# Autodesk Inventor assembly: enc-BackPanel Top - Assembly
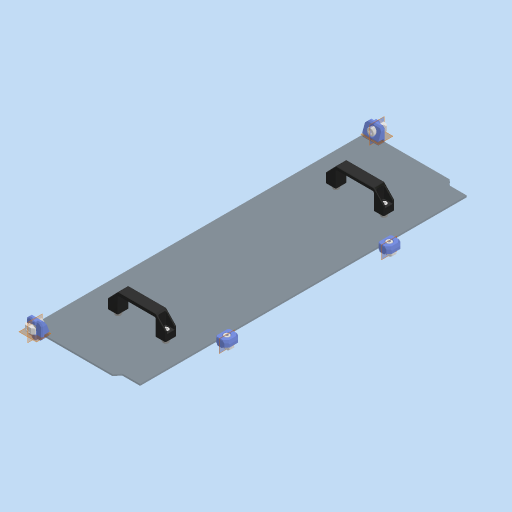
[picture p0: Inventor's stored thumbnail of the model, 512x512]
Saved by Autodesk Inventor 2023.2 (Build 272271000, 271)
## iProperties
Created: 2023-12-04
Part Number: enc-BackPanel Top - Assembly
Document SubType Name: Assembly
Designer: Nils Bade
Author: Nils Bade
## Documents named in this file (7)
- C:\Users\nilsb\Documents\Inventor\Projektarbeit-Bade\Enclosure\enc-BackPanel Top - Assembly.iam
- C:\Users\nilsb\Documents\Inventor\Projektarbeit-Bade\Enclosure\enc-BackPanel Top.ipt
- C:\Users\nilsb\Documents\Inventor\Projektarbeit-Bade\Enclosure\V-Slot Door Handle v1.ipt
- C:\Users\nilsb\Documents\Inventor\Projektarbeit-Bade\Schrauben\Cap Head Screw M6x16 - DIN912.ipt
- C:\Users\nilsb\Documents\Inventor\Projektarbeit-Bade\RatRig_Standards\Hex Locking Nut - M6 v2.ipt
- C:\Users\nilsb\Documents\Inventor\Projektarbeit-Bade\Enclosure\Panel Mount Vertical Support for 4040 - Assembly.iam
- C:\Users\nilsb\Documents\Inventor\Projektarbeit-Bade\Enclosure\Panel Mount Vertical Guide for 4040 - Assembly.iam
## Components (15 placed, 6 different names)
1. enc-BackPanel Top for 4040:1 — Passend:1, Passend:2, Passend:3, Passend:4, Passend:5, Passend:6, Passend:17, Passend:18, Passend:19, Passend:20, Passend:21, Passend:22, Fluchtend:1, Fluchtend:2, Passend:23, Passend:24, Fluchtend:3, Fluchtend:4, Passend:25, Passend:26
2. V-Slot Door Handle v1:1 — Passend:4, Passend:5, Passend:6, Passend:7, Passend:8, Passend:11, Passend:12
3. V-Slot Door Handle v1:2 — Passend:1, Passend:2, Passend:3, Passend:9, Einfügen:1, Passend:10
4. Cap Head Screw M6x16 - DIN912:1 — Passend:7, Passend:12, Passend:14
5. Cap Head Screw M6x16 - DIN912:2 — Passend:8, Passend:11, Passend:13
6. Cap Head Screw M6x16 - DIN912:3 — Passend:9, Passend:10, Passend:15
7. Cap Head Screw M6x16 - DIN912:4 — Einfügen:1, Passend:16
8. Hex Locking Nut - M6 v2:1 — Passend:13, Passend:17
9. Hex Locking Nut - M6 v2:2 — Passend:14, Passend:18
10. Hex Locking Nut - M6 v2:3 — Passend:15, Passend:20
11. Hex Locking Nut - M6 v2:4 — Passend:16, Passend:19
12. Panel Mount Vertical Support for 4040 - Assembly:1 [sub-assembly] — Passend:21, Fluchtend:2, Fluchtend:4, Fluchtend:5
13. Panel Mount Vertical Support for 4040 - Assembly:2 [sub-assembly] — Passend:22, Fluchtend:1, Fluchtend:3, Passend:27
14. Panel Mount Vertical Guide for 4040 - Assembly:1 [sub-assembly] — Passend:25, Passend:26, Fluchtend:5
15. Panel Mount Vertical Guide for 4040 - Assembly:2 [sub-assembly] — Passend:23, Passend:24, Passend:27
## Relationships (33: Mate 27, Flush 5, Insert 1)
- Passend:1 [Mate]: enc-BackPanel Top for 4040:1 ↔ V-Slot Door Handle v1:2
- Passend:2 [Mate]: enc-BackPanel Top for 4040:1 ↔ V-Slot Door Handle v1:2
- Passend:3 [Mate]: enc-BackPanel Top for 4040:1 ↔ V-Slot Door Handle v1:2
- Passend:4 [Mate]: enc-BackPanel Top for 4040:1 ↔ V-Slot Door Handle v1:1
- Passend:5 [Mate]: enc-BackPanel Top for 4040:1 ↔ V-Slot Door Handle v1:1
- Passend:6 [Mate]: enc-BackPanel Top for 4040:1 ↔ V-Slot Door Handle v1:1
- Passend:7 [Mate]: V-Slot Door Handle v1:1 ↔ Cap Head Screw M6x16 - DIN912:1
- Passend:8 [Mate]: V-Slot Door Handle v1:1 ↔ Cap Head Screw M6x16 - DIN912:2
- Passend:9 [Mate]: V-Slot Door Handle v1:2 ↔ Cap Head Screw M6x16 - DIN912:3
- Einfügen:1 [Insert]: V-Slot Door Handle v1:2 ↔ Cap Head Screw M6x16 - DIN912:4
- Passend:10 [Mate]: V-Slot Door Handle v1:2 ↔ Cap Head Screw M6x16 - DIN912:3
- Passend:11 [Mate]: V-Slot Door Handle v1:1 ↔ Cap Head Screw M6x16 - DIN912:2
- Passend:12 [Mate]: V-Slot Door Handle v1:1 ↔ Cap Head Screw M6x16 - DIN912:1
- Passend:13 [Mate]: Cap Head Screw M6x16 - DIN912:2 ↔ Hex Locking Nut - M6 v2:1
- Passend:14 [Mate]: Cap Head Screw M6x16 - DIN912:1 ↔ Hex Locking Nut - M6 v2:2
- Passend:15 [Mate]: Cap Head Screw M6x16 - DIN912:3 ↔ Hex Locking Nut - M6 v2:3
- Passend:16 [Mate]: Cap Head Screw M6x16 - DIN912:4 ↔ Hex Locking Nut - M6 v2:4
- Passend:17 [Mate]: enc-BackPanel Top for 4040:1 ↔ Hex Locking Nut - M6 v2:1
- Passend:18 [Mate]: enc-BackPanel Top for 4040:1 ↔ Hex Locking Nut - M6 v2:2
- Passend:19 [Mate]: enc-BackPanel Top for 4040:1 ↔ Hex Locking Nut - M6 v2:4
- Passend:20 [Mate]: enc-BackPanel Top for 4040:1 ↔ Hex Locking Nut - M6 v2:3
- Passend:21 [Mate]: enc-BackPanel Top for 4040:1 ↔ Panel Mount Vertical Support for 4040 - Assembly:1
- Passend:22 [Mate]: enc-BackPanel Top for 4040:1 ↔ Panel Mount Vertical Support for 4040 - Assembly:2
- Fluchtend:1 [Flush] (150 mm): enc-BackPanel Top for 4040:1 ↔ Panel Mount Vertical Support for 4040 - Assembly:2
- Fluchtend:2 [Flush] (150 mm): enc-BackPanel Top for 4040:1 ↔ Panel Mount Vertical Support for 4040 - Assembly:1
- Passend:23 [Mate]: enc-BackPanel Top for 4040:1 ↔ Panel Mount Vertical Guide for 4040 - Assembly:2
- Passend:24 [Mate] (2 mm): enc-BackPanel Top for 4040:1 ↔ Panel Mount Vertical Guide for 4040 - Assembly:2
- Fluchtend:3 [Flush]: enc-BackPanel Top for 4040:1 ↔ Panel Mount Vertical Support for 4040 - Assembly:2
- Fluchtend:4 [Flush]: enc-BackPanel Top for 4040:1 ↔ Panel Mount Vertical Support for 4040 - Assembly:1
- Passend:25 [Mate]: enc-BackPanel Top for 4040:1 ↔ Panel Mount Vertical Guide for 4040 - Assembly:1
- Passend:26 [Mate] (2 mm): enc-BackPanel Top for 4040:1 ↔ Panel Mount Vertical Guide for 4040 - Assembly:1
- Passend:27 [Mate] (190 mm): Panel Mount Vertical Support for 4040 - Assembly:2 ↔ Panel Mount Vertical Guide for 4040 - Assembly:2
- Fluchtend:5 [Flush] (190 mm): Panel Mount Vertical Support for 4040 - Assembly:1 ↔ Panel Mount Vertical Guide for 4040 - Assembly:1
